# Autodesk Inventor assembly: Assembly1
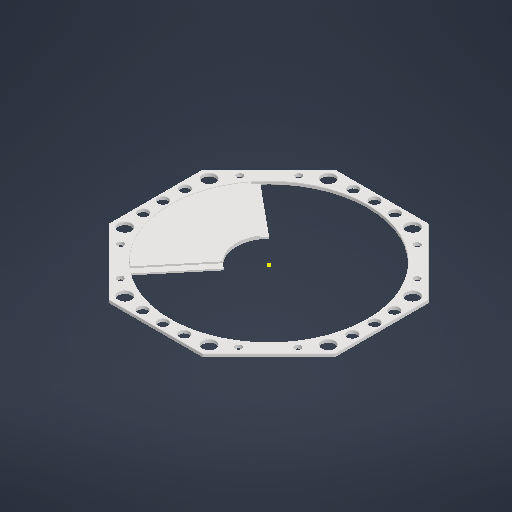
[picture p0: Inventor's stored thumbnail of the model, 512x512]
Saved by Autodesk Inventor 2026.2 (Build 302298000, 298)
## iProperties
Created: 2025-12-09
Part Number: Assembly1
Document SubType Name: Assembly
Designer: Thoma
Author: Thoma
## Documents named in this file (3)
- C:\Users\Thoma\OneDrive\Desktop\Inventor\Quarter_Open\Version_1\Assembly1.iam
- C:\Users\Thoma\OneDrive\Desktop\Inventor\Quarter_Open\Version_1\Telescope_End.ipt
- C:\Users\Thoma\OneDrive\Desktop\Inventor\Quarter_Open\Version_1\Part1.ipt
## Components (2 placed, 2 different names)
1. Telescope_End:1 — Mate:1, Flush:1
2. Part1:1 — Mate:1, Flush:1
## Relationships (2: Mate 1, Flush 1)
- Mate:1: Telescope_End:1 ↔ Part1:1
- Flush:1: Telescope_End:1 ↔ Part1:1
